# Autodesk Inventor assembly: CN2596-2
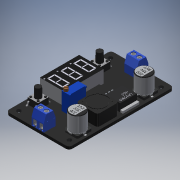
[picture p0: Inventor's stored thumbnail of the model, 180x180]
Saved by Autodesk Inventor 2019 (Build 230136000, 136)
## iProperties
Created: 2016-12-15
Part Number: CN2596-2
Document SubType Name: Assembly
Designer: close
Sending System: Autodesk Inventor 2016
Preprocessor: ST-DEVELOPER v16.1
Title: C:\Users\rdusak\Documents\Inventor\Machine_for_bending_wire\STEP\CN2596-2.stp
Author: RDusak
## Documents named in this file (9)
- C:\Users\close\Desktop\CAD BARC-ROAR\Dependencies\Drok Step Down\CN2596-2.iam
- C:\Users\close\Desktop\CAD BARC-ROAR\Dependencies\Drok Step Down\LM2596S-ADJ.ipt
- C:\Users\close\Desktop\CAD BARC-ROAR\Dependencies\Drok Step Down\3631AH-6.8P.ipt
- C:\Users\close\Desktop\CAD BARC-ROAR\Dependencies\Drok Step Down\Trimpot_3296W.ipt
- C:\Users\close\Desktop\CAD BARC-ROAR\Dependencies\Drok Step Down\CAPAE-D8.0x10.2.ipt
- C:\Users\close\Desktop\CAD BARC-ROAR\Dependencies\Drok Step Down\Drok Step Down PCB.ipt
- C:\Users\close\Desktop\CAD BARC-ROAR\Dependencies\Drok Step Down\Screw Terminal Block 3.5mm Blue 2-way.ipt
- C:\Users\close\Desktop\CAD BARC-ROAR\Dependencies\Tactile Switches\Tactal Switch - SMD (6mmx 6mmx 9mm) - Marked.ipt
- C:\Users\close\Desktop\CAD BARC-ROAR\Dependencies\Drok Step Down\coil.ipt
## Components (11 placed, 8 different names)
1. LM2596S-ADJ:1 — Mate:5, Mate:16, Flush:12
2. 3631AH-6.8P:1 — Mate:1, Flush:5, Flush:6, Mate:13, Mate:14, Mate:15, Flush:9
3. Trimpot_3296W:1 — Mate:9, Mate:15, Flush:9
4. CAPAE-D8.0x10.2:1 — Mate:6, Flush:13, Flush:15, Flush:16
5. CAPAE-D8.0x10.2:2 — Mate:4, Flush:13, Flush:14
6. Drok Step Down PCB:1 — Mate:1, Mate:4, Mate:5, Mate:6, Mate:7, Mate:8, Flush:1, Flush:2, Mate:9, Mate:10, Mate:11, Flush:4, Flush:5, Mate:12, Flush:6, Flush:7, Flush:8, Flush:10, Flush:11, Flush:12, Flush:14, Flush:15, Flush:16
7. Screw Terminal Block 3.5mm Blue 2-way:1 — Mate:7, Flush:2, Flush:7
8. Screw Terminal Block 3.5mm Blue 2-way:2 — Mate:8, Flush:1, Flush:8
9. Tactal Switch - SMD (6mmx 6mmx 9mm) - Marked:1 — Mate:10, Flush:3, Flush:4, Mate:14
10. Tactal Switch - SMD (6mmx 6mmx 9mm) - Marked:2 — Mate:11, Flush:3, Mate:13
11. coil:1 — Mate:12, Flush:10, Flush:11, Mate:16
## Relationships (30: Flush 16, Mate 14)
- Mate:1: 3631AH-6.8P:1 ↔ Drok Step Down PCB:1
- Mate:4: CAPAE-D8.0x10.2:2 ↔ Drok Step Down PCB:1
- Mate:5: LM2596S-ADJ:1 ↔ Drok Step Down PCB:1
- Mate:6: CAPAE-D8.0x10.2:1 ↔ Drok Step Down PCB:1
- Mate:7: Drok Step Down PCB:1 ↔ Screw Terminal Block 3.5mm Blue 2-way:1
- Mate:8: Drok Step Down PCB:1 ↔ Screw Terminal Block 3.5mm Blue 2-way:2
- Flush:1: Drok Step Down PCB:1 ↔ Screw Terminal Block 3.5mm Blue 2-way:2
- Flush:2: Drok Step Down PCB:1 ↔ Screw Terminal Block 3.5mm Blue 2-way:1
- Mate:9: Trimpot_3296W:1 ↔ Drok Step Down PCB:1
- Mate:10: Drok Step Down PCB:1 ↔ Tactal Switch - SMD (6mmx 6mmx 9mm) - Marked:1
- Mate:11: Drok Step Down PCB:1 ↔ Tactal Switch - SMD (6mmx 6mmx 9mm) - Marked:2
- Flush:3: Tactal Switch - SMD (6mmx 6mmx 9mm) - Marked:1 ↔ Tactal Switch - SMD (6mmx 6mmx 9mm) - Marked:2
- Flush:4 (2.75 mm): Drok Step Down PCB:1 ↔ Tactal Switch - SMD (6mmx 6mmx 9mm) - Marked:1
- Flush:5 (0.3 mm): 3631AH-6.8P:1 ↔ Drok Step Down PCB:1
- Mate:12: Drok Step Down PCB:1 ↔ coil:1
- Flush:6 (19 mm): 3631AH-6.8P:1 ↔ Drok Step Down PCB:1
- Flush:7 (14.5 mm): Drok Step Down PCB:1 ↔ Screw Terminal Block 3.5mm Blue 2-way:1
- Flush:8 (14.5 mm): Drok Step Down PCB:1 ↔ Screw Terminal Block 3.5mm Blue 2-way:2
- Mate:13 (3.25 mm): 3631AH-6.8P:1 ↔ Tactal Switch - SMD (6mmx 6mmx 9mm) - Marked:2
- Mate:14 (3.5 mm): 3631AH-6.8P:1 ↔ Tactal Switch - SMD (6mmx 6mmx 9mm) - Marked:1
- Mate:15 (1.4 mm): 3631AH-6.8P:1 ↔ Trimpot_3296W:1
- Flush:9 (-3 mm): 3631AH-6.8P:1 ↔ Trimpot_3296W:1
- Flush:10 (18 mm): Drok Step Down PCB:1 ↔ coil:1
- Flush:11 (1.7 mm): Drok Step Down PCB:1 ↔ coil:1
- Mate:16 (1.8 mm): LM2596S-ADJ:1 ↔ coil:1
- Flush:12 (1.25 mm): LM2596S-ADJ:1 ↔ Drok Step Down PCB:1
- Flush:13: CAPAE-D8.0x10.2:1 ↔ CAPAE-D8.0x10.2:2
- Flush:14 (6.85 mm): CAPAE-D8.0x10.2:2 ↔ Drok Step Down PCB:1
- Flush:15 (6.45 mm): CAPAE-D8.0x10.2:1 ↔ Drok Step Down PCB:1
- Flush:16 (1.65 mm): CAPAE-D8.0x10.2:1 ↔ Drok Step Down PCB:1
